# Autodesk Inventor assembly: joint
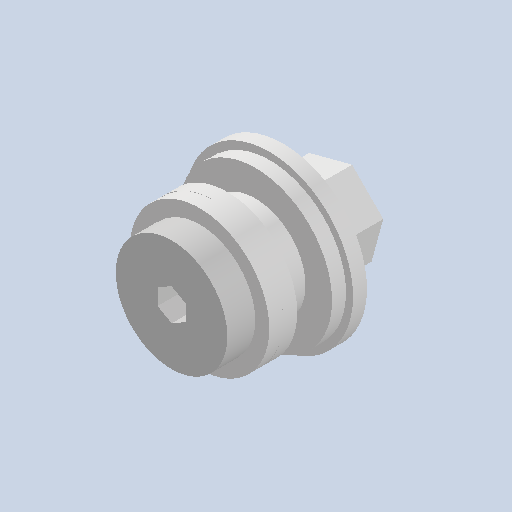
[picture p0: Inventor's stored thumbnail of the model, 512x512]
Saved by Autodesk Inventor 2022 (Build 260153000, 153)
## iProperties
Created: 2022-10-13
Part Number: joint
Document SubType Name: Assembly
Designer: haya
Author: haya
## Documents named in this file (7)
- C:\Users\haya\Documents\GitHub\OpenPlatform_ver3_0 - コピー\joint.iam
- C:\Users\haya\Documents\GitHub\OpenPlatform_ver3_0 - コピー\S3-15-3W.ipt
- C:\Users\haya\Documents\GitHub\OpenPlatform_ver3_0 - コピー\80F-0503.ipt
- C:\Users\haya\Documents\GitHub\OpenPlatform_ver3_0 - コピー\AAW-0510-10.ipt
- C:\Users\haya\Documents\GitHub\OpenPlatform_ver3_0 - コピー\LL-7211-10.ipt
- C:\Users\haya\Documents\GitHub\OpenPlatform_ver3_0 - コピー\DBB3-5-5.ipt
- C:\Users\haya\Documents\GitHub\OpenPlatform_ver3_0 - コピー\UUW-0312-10H.ipt
## Components (6 placed, 6 different names)
1. S3-15-3W:1
2. 80F-0503:1
3. AAW-0510-10:1
4. LL-7211-10:1
5. DBB3-5-5:1
6. UUW-0312-10H:1
## Relationships (5: Insert 5)
- [Insert]: 80F-0503:1 ↔ AAW-0510-10:1
- [Insert]: 80F-0503:1 ↔ LL-7211-10:1
- [Insert]: 80F-0503:1 ↔ UUW-0312-10H:1
- [Insert] (2 mm): S3-15-3W:1 ↔ UUW-0312-10H:1
- [Insert]: AAW-0510-10:1 ↔ DBB3-5-5:1
## Named parameters: d85_d72_d61_d34 = 0 mm, d87_d74_d66 = 0 mm
